# Autodesk Inventor assembly: Servo
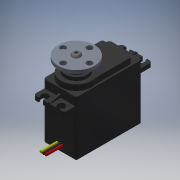
[picture p0: Inventor's stored thumbnail of the model, 180x180]
Saved by Autodesk Inventor 2017 (Build 210142000, 142)
## iProperties
Created: 2013-08-31
Part Number: Servo
Document SubType Name: Assembly
Designer: sfreisem-kirov
Sending System: Autodesk Inventor 2014
Preprocessor: ST-DEVELOPER v15.2
Title: C:\Users\Kyle\Documents\Tetrix_Kit_FTC\tetrix_739197_2012.stp
Author: Kyle
## Documents named in this file (4)
- C:\Users\sfreisem-kirov\Documents\GitHub\ftc_app\Parts\phoneHolder\Servo.iam
- C:\Users\sfreisem-kirov\Documents\GitHub\ftc_app\Parts\phoneHolder\TETRIX_739197_SERVO_2012.ipt
- C:\Users\sfreisem-kirov\Documents\GitHub\ftc_app\Parts\phoneHolder\TETRIX_739197_METAL_HORN_2012.ipt
- C:\Users\sfreisem-kirov\Documents\GitHub\ftc_app\Parts\phoneHolder\TETRIX_739197_SCREW_2012.ipt
## Components (3 placed, 3 different names)
1. TETRIX_739197_SERVO_2012:1 — Mate:2, Mate:4
2. TETRIX_739197_METAL_HORN_2012:1 — Mate:1, Mate:3, Mate:4
3. TETRIX_739197_SCREW_2012:1 — Mate:1, Mate:2, Mate:3
## Relationships (4: Mate 4)
- Mate:1: TETRIX_739197_METAL_HORN_2012:1 ↔ TETRIX_739197_SCREW_2012:1
- Mate:2: TETRIX_739197_SERVO_2012:1 ↔ TETRIX_739197_SCREW_2012:1
- Mate:3: TETRIX_739197_METAL_HORN_2012:1 ↔ TETRIX_739197_SCREW_2012:1
- Mate:4: TETRIX_739197_SERVO_2012:1 ↔ TETRIX_739197_METAL_HORN_2012:1
